# Autodesk Inventor assembly: Beaker glass - top connector
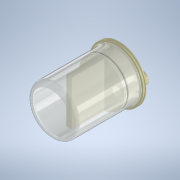
[picture p0: Inventor's stored thumbnail of the model, 180x180]
Saved by Autodesk Inventor 2020.3 (Build 243373000, 373)
## iProperties
Created: 2020-08-07
Part Number: Beaker glass - top connector
Document SubType Name: Assembly
Designer: Bruno
Author: Bruno
## Documents named in this file (13)
- C:\Users\Bruno\Desktop\CAD GH3\Inventor\Ventilation pipeline\Beaker glass - top connector.iam
- C:\Users\Bruno\Desktop\CAD GH3\Inventor\Ventilation pipeline\Beaker glass - top connector\Beaker glass 600ml, diam_ 90mm.ipt
- C:\Users\Bruno\Desktop\CAD GH3\Inventor\Ventilation pipeline\Beaker glass - top connector\Top lid body.ipt
- C:\Users\Bruno\Desktop\CAD GH3\Inventor\Ventilation pipeline\Beaker glass - top connector\Paddle.ipt
- C:\Users\Bruno\Desktop\CAD GH3\Inventor\Ventilation pipeline\Beaker glass - top connector\Oring 2-007.ipt
- C:\Users\Bruno\Desktop\CAD GH3\Inventor\Ventilation pipeline\Beaker glass - top connector\DIN912 M4x0.7x16-8.8 socket head screw.ipt
- C:\Users\Bruno\Desktop\CAD GH3\Inventor\Ventilation pipeline\Beaker glass - top connector\Oring 2-026.ipt
- C:\Users\Bruno\Desktop\CAD GH3\Inventor\Ventilation pipeline\Beaker glass - top connector\Oring 2-019.ipt
- C:\Users\Bruno\Desktop\CAD GH3\Inventor\Ventilation pipeline\Beaker glass - top connector\Oring 2-151_D.ipt
- C:\Users\Bruno\Desktop\CAD GH3\Inventor\Ventilation pipeline\Beaker glass - top connector\Corrugated tube-top lid connector.ipt
- C:\Users\Bruno\Desktop\CAD GH3\Inventor\Ventilation pipeline\Beaker glass - top connector\Heated tube-top lid connector.ipt
- C:\Users\Bruno\Desktop\CAD GH3\Inventor\Ventilation pipeline\Beaker glass - top connector\Oring 2-018_D.ipt
- C:\Users\Bruno\Desktop\CAD GH3\Inventor\Ventilation pipeline\Beaker glass - top connector\Oring 2-022.ipt
## Components (12 placed, 12 different names)
1. Beaker glass 600ml, diam_ 90mm:1 — Cylindrical:31
2. Top lid body:1 — Cylindrical:22, Cylindrical:23, Rigid:1, Cylindrical:25, Cylindrical:26, Cylindrical:27, Cylindrical:28, Cylindrical:31
3. Paddle:1 — Cylindrical:22
4. Oring 2-007:1 — Cylindrical:23, Cylindrical:24
5. DIN912 M4x0.7x16-8.8 socket head screw:1 — Cylindrical:24
6. Oring 2-026:1 — Rigid:1
7. Oring 2-019:1 — Cylindrical:25
8. Oring 2-151_D:1 — Cylindrical:26
9. Corrugated tube-top lid connector:1 — Cylindrical:27, Cylindrical:30
10. Heated tube-top lid connector:1 — Cylindrical:28, Cylindrical:29
11. Oring 2-018_D:1 — Cylindrical:30
12. Oring 2-022:1 — Cylindrical:29
## Relationships (11: CylindricalJoint 10, WeldJoint 1)
- Cylindrical:22: Top lid body:1 ↔ Paddle:1
- Cylindrical:23: Top lid body:1 ↔ Oring 2-007:1
- Cylindrical:24: Oring 2-007:1 ↔ DIN912 M4x0.7x16-8.8 socket head screw:1
- Rigid:1 [WeldJoint] (-1.5 mm): Top lid body:1 ↔ Oring 2-026:1
- Cylindrical:25: Top lid body:1 ↔ Oring 2-019:1
- Cylindrical:26: Top lid body:1 ↔ Oring 2-151_D:1
- Cylindrical:27: Top lid body:1 ↔ Corrugated tube-top lid connector:1
- Cylindrical:28: Top lid body:1 ↔ Heated tube-top lid connector:1
- Cylindrical:29: Heated tube-top lid connector:1 ↔ Oring 2-022:1
- Cylindrical:30: Corrugated tube-top lid connector:1 ↔ Oring 2-018_D:1
- Cylindrical:31: Beaker glass 600ml, diam_ 90mm:1 ↔ Top lid body:1
